# Autodesk Inventor assembly: SolderingStation
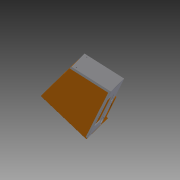
[picture p0: Inventor's stored thumbnail of the model, 180x180]
Saved by Autodesk Inventor 2015 SP2 (Build 190223200, 223)
## iProperties
Created: 2018-06-26
Part Number: SolderingStation
Document SubType Name: Assembly
Designer: loetscher_l
Author: loetscher_l
## Documents named in this file (3)
- K:\020_Beamline\210_Development\520_SolderStation\Github\3D-elements\SolderingStation.iam
- K:\020_Beamline\210_Development\520_SolderStation\Github\3D-elements\SolderingStation.ipt
- K:\020_Beamline\210_Development\520_SolderStation\Github\3D-elements\Top.ipt
## Components (2 placed, 2 different names)
1. SolderingStation:1 — Einfügen:1, Fluchtend:1
2. Top:1 — Einfügen:1, Fluchtend:1
## Relationships (2: Insert 1, Flush 1)
- Einfügen:1 [Insert]: SolderingStation:1 ↔ Top:1
- Fluchtend:1 [Flush]: SolderingStation:1 ↔ Top:1
